# Autodesk Inventor assembly: Eslabon_3
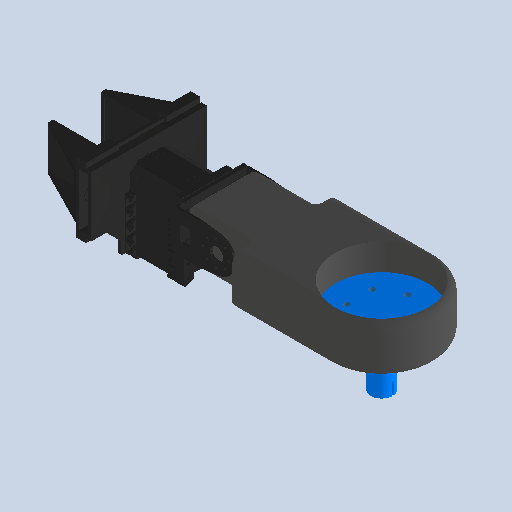
[picture p0: Inventor's stored thumbnail of the model, 512x512]
Saved by Autodesk Inventor 2024 (Build 280153000, 153)
## iProperties
Created: 2022-06-07
Part Number: Eslabon_3
Document SubType Name: Assembly
Designer: Alcatraz
Author: Alcatraz
## Documents named in this file (4)
- C:\Users\Alcatraz\Desktop\TESIS-actual\Lista_Piezas_MovPlano_21Junio\Lista_Piezas\Eslabon_3.iam
- C:\Users\Alcatraz\Desktop\TESIS-actual\Lista_Piezas_MovPlano_21Junio\Lista_Piezas\Eje_01.ipt
- C:\Users\Alcatraz\Desktop\TESIS-actual\Lista_Piezas_MovPlano_21Junio\Lista_Piezas\Es_03.ipt
- C:\Users\Alcatraz\Desktop\TESIS-actual\GRIPPER_M.iam
## Components (3 placed, 3 different names)
1. Eje_01:1 — Coincidencia:1, Coincidencia:2, Coincidencia:3
2. Es_03:1 — Coincidencia:1, Coincidencia:2, Coincidencia:3, Coincidencia:4, Coincidencia:5, Coincidencia:6
3. GRIPPER_M:1 [sub-assembly] — Coincidencia:4, Coincidencia:5, Coincidencia:6
## Relationships (6: Mate 6)
- Coincidencia:1 [Mate]: Eje_01:1 ↔ Es_03:1
- Coincidencia:2 [Mate]: Eje_01:1 ↔ Es_03:1
- Coincidencia:3 [Mate]: Eje_01:1 ↔ Es_03:1
- Coincidencia:4 [Mate]: Es_03:1 ↔ GRIPPER_M:1
- Coincidencia:5 [Mate]: Es_03:1 ↔ GRIPPER_M:1
- Coincidencia:6 [Mate]: Es_03:1 ↔ GRIPPER_M:1
